# Autodesk Inventor assembly: Bearing Assembly Arms
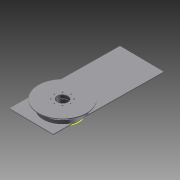
[picture p0: Inventor's stored thumbnail of the model, 180x180]
Saved by Autodesk Inventor 2015 (Build 190159000, 159)
## iProperties
Created: 2015-01-18
Part Number: Bearing Assembly Arms
Document SubType Name: Assembly
Designer: chapale16
Author: chapale16
## Documents named in this file (4)
- \\lhssvr02\Homedirs\Robotics Club\CAD Model 2015\Bearing Assembly Arms.iam
- \\lhssvr02\Homedirs\Robotics Club\CAD Model 2015\bearing plate.ipt
- \\lhssvr02\Homedirs\Robotics Club\CAD Model 2015\S25-60L Aluminum Sprocket (am-0237).ipt
- \\lhssvr02\Homedirs\Robotics Club\CAD Model 2015\Game Components\The Tote Collector-Arms\Imported Components\PRT_01_30_1\PRT_01_30_1.iam
## Components (3 placed, 3 different names)
1. PRT_01_30_1:1 [sub-assembly] — Mate:3, Mate:4
2. S25-60L Aluminum Sprocket (am-0237):1
3. bearing plate:1 — Mate:3, Mate:4
## Relationships (4: Mate 4)
- [Mate]: PRT_01_30_1:1 ↔ S25-60L Aluminum Sprocket (am-0237):1
- [Mate]: PRT_01_30_1:1 ↔ S25-60L Aluminum Sprocket (am-0237):1
- Mate:3: PRT_01_30_1:1 ↔ bearing plate:1
- Mate:4: PRT_01_30_1:1 ↔ bearing plate:1
